# Autodesk Inventor assembly: タミヤダンパー1
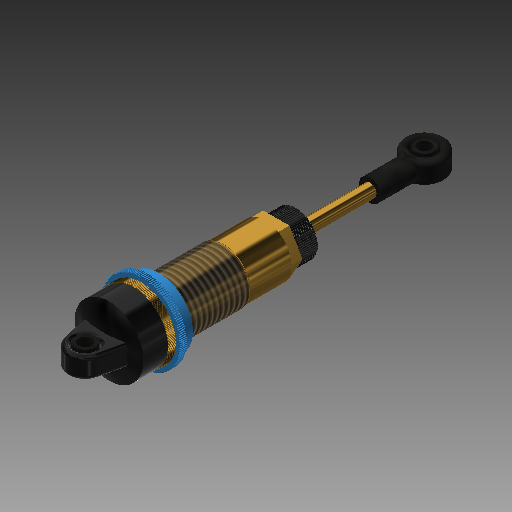
[picture p0: Inventor's stored thumbnail of the model, 512x512]
Saved by Autodesk Inventor 2020 (Build 240168000, 168)
## iProperties
Part Number: タミヤダンパー1
Material: 一般
Document SubType Name: Assembly
Designer: 雪村
Mass: 29.9788 g
Surface Area: 59.981 cm^2
Volume: 5.28575 cm^3
Density: 5.67163 g/cm^3
Author: 雪村
## Documents named in this file (9)
- C:\Users\white\Documents\SRDC\SRDC\Inventor_2017\2018年機体\パーツ\タミヤダンパー.iam
- C:\Users\white\Documents\SRDC\SRDC\Inventor_2017\2018年機体\パーツ\タミヤダンパー1.ipt
- C:\Users\white\Documents\SRDC\SRDC\Inventor_2017\2018年機体\パーツ\タミヤダンパー2.ipt
- C:\Users\white\Documents\SRDC\SRDC\Inventor_2017\2018年機体\パーツ\タミヤダンパー3.ipt
- C:\Users\white\Documents\SRDC\SRDC\Inventor_2017\2018年機体\パーツ\タミヤダンパー4.ipt
- C:\Users\white\Documents\SRDC\SRDC\Inventor_2017\2018年機体\パーツ\タミヤダンパー6.ipt
- C:\Users\white\Documents\SRDC\SRDC\Inventor_2017\2018年機体\パーツ\タミヤダンパー5.ipt
- C:\Users\white\Documents\SRDC\SRDC\Inventor_2017\2018年機体\パーツ\タミヤダンパー7.ipt
- C:\Users\white\Documents\SRDC\SRDC\Inventor_2017\2018年機体\パーツ\タミヤダンパー8.ipt
## Components (9 placed, 8 different names)
1. タミヤダンパー1:1 — 挿入:1, ボール:2, フラッシュ:1
2. タミヤダンパー2:1 — 挿入:1, メイト:1, 挿入:4, 円柱状:1, 角度:1
3. タミヤダンパー3:1 — 挿入:3, 挿入:4
4. タミヤダンパー4:1 — メイト:1
5. タミヤダンパー6:1 — 挿入:3
6. タミヤダンパー5:1 — 円柱状:1, 挿入:5
7. タミヤダンパー7:1 — ボール:1, 挿入:5, 正接:1
8. タミヤダンパー8:1 — ボール:2, フラッシュ:1
9. タミヤダンパー8:2 — ボール:1, 正接:1, 角度:1
## Relationships (11: Insert 4, BallJoint 2, Mate 1, CylindricalJoint 1, Flush 1, Tangent 1, Angle 1)
- 挿入:1 [Insert]: タミヤダンパー1:1 ↔ タミヤダンパー2:1
- メイト:1 [Mate]: タミヤダンパー2:1 ↔ タミヤダンパー4:1
- 挿入:3 [Insert]: タミヤダンパー3:1 ↔ タミヤダンパー6:1
- ボール:1 [BallJoint]: タミヤダンパー7:1 ↔ タミヤダンパー8:2
- 挿入:4 [Insert]: タミヤダンパー2:1 ↔ タミヤダンパー3:1
- 円柱状:1 [CylindricalJoint]: タミヤダンパー2:1 ↔ タミヤダンパー5:1
- 挿入:5 [Insert]: タミヤダンパー5:1 ↔ タミヤダンパー7:1
- ボール:2 [BallJoint]: タミヤダンパー1:1 ↔ タミヤダンパー8:1
- フラッシュ:1 [Flush]: タミヤダンパー1:1 ↔ タミヤダンパー8:1
- 正接:1 [Tangent]: タミヤダンパー7:1 ↔ タミヤダンパー8:2
- 角度:1 [Angle] (0 deg): タミヤダンパー2:1 ↔ タミヤダンパー8:2
